# Autodesk Inventor assembly: Assembly1
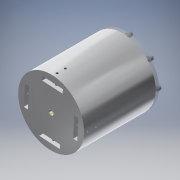
[picture p0: Inventor's stored thumbnail of the model, 180x180]
Saved by Autodesk Inventor 2016 (Build 200138000, 138)
## iProperties
Created: 2016-07-05
Part Number: Assembly1
Document SubType Name: Assembly
Designer: Andres
Author: Andres
## Documents named in this file (5)
- \\Mac\Home\Documents\repositorios\BoreholeCamera\CAD_Probe\Enclosure\Assembly\Assembly1.iam
- \\Mac\Home\Documents\repositorios\BoreholeCamera\CAD_Probe\Enclosure\Parts\Enclosure.ipt
- \\Mac\Home\Documents\repositorios\BoreholeCamera\CAD_Probe\Enclosure\Parts\Cover.ipt
- \\Mac\Home\Documents\repositorios\BoreholeCamera\CAD_Probe\Enclosure\Assembly\Assembly1\Design Accelerator\O-Ring4.iam
- Z:\Documents\repositorios\BoreholeCamera\CAD_Probe\Enclosure\Parts\TYPE 316 SS SOCKET HEAD CAP SCREW.ipt
## Components (11 placed, 4 different names)
1. Enclosure:1 — Mate:1, Mate:2, Rotational:5
2. Cover:1 — Rotational:5, Rotational:6, Rotational:7, Rotational:8, Rotational:9, Rotational:10, Rotational:11, Rotational:12, Rotational:13
3. O-Ring:1 [sub-assembly] — Mate:1, Mate:2
4. TYPE 316 SS SOCKET HEAD CAP SCREW:2 — Rotational:6
5. TYPE 316 SS SOCKET HEAD CAP SCREW:4 — Rotational:8
6. TYPE 316 SS SOCKET HEAD CAP SCREW:6 — Rotational:7
7. TYPE 316 SS SOCKET HEAD CAP SCREW:7 — Rotational:9
8. TYPE 316 SS SOCKET HEAD CAP SCREW:8 — Rotational:10
9. TYPE 316 SS SOCKET HEAD CAP SCREW:9 — Rotational:11
10. TYPE 316 SS SOCKET HEAD CAP SCREW:11 — Rotational:12
11. TYPE 316 SS SOCKET HEAD CAP SCREW:12 — Rotational:13
## Relationships (11: RevoluteJoint 9, Mate 2)
- Mate:1: Enclosure:1 ↔ O-Ring:1
- Mate:2: Enclosure:1 ↔ O-Ring:1
- Rotational:5 [RevoluteJoint]: Enclosure:1 ↔ Cover:1
- Rotational:6 [RevoluteJoint]: Cover:1 ↔ TYPE 316 SS SOCKET HEAD CAP SCREW:2
- Rotational:7 [RevoluteJoint]: Cover:1 ↔ TYPE 316 SS SOCKET HEAD CAP SCREW:6
- Rotational:8 [RevoluteJoint]: Cover:1 ↔ TYPE 316 SS SOCKET HEAD CAP SCREW:4
- Rotational:9 [RevoluteJoint]: Cover:1 ↔ TYPE 316 SS SOCKET HEAD CAP SCREW:7
- Rotational:10 [RevoluteJoint]: Cover:1 ↔ TYPE 316 SS SOCKET HEAD CAP SCREW:8
- Rotational:11 [RevoluteJoint]: Cover:1 ↔ TYPE 316 SS SOCKET HEAD CAP SCREW:9
- Rotational:12 [RevoluteJoint]: Cover:1 ↔ TYPE 316 SS SOCKET HEAD CAP SCREW:11
- Rotational:13 [RevoluteJoint]: Cover:1 ↔ TYPE 316 SS SOCKET HEAD CAP SCREW:12
